# Autodesk Inventor assembly: outsideHand
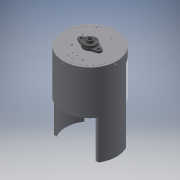
[picture p0: Inventor's stored thumbnail of the model, 180x180]
Saved by Autodesk Inventor 2016 (Build 200138000, 138)
## iProperties
Created: 2016-11-12
Part Number: outsideHand
Material: 一般
Document SubType Name: Assembly
Designer: Daisuke
Author: Daisuke
## Documents named in this file (5)
- C:\Users\Daisuke\Documents\GitHub\CAD\Hand\ver1\outsideHand.iam
- C:\Users\Daisuke\Documents\GitHub\CAD\Hand\ver1\UFL08 -Housing.ipt
- C:\Users\Daisuke\Documents\GitHub\CAD\Hand\ver1\UltrasonicDistanceSencor.ipt
- C:\Users\Daisuke\Documents\GitHub\CAD\Hand\ver1\outsideBottom.ipt
- C:\Users\Daisuke\Documents\GitHub\CAD\Hand\ver1\outsideCover.iam
## Components (4 placed, 4 different names)
1. UFL08 -Housing:1 — 挿入:2, 挿入:3
2. UltrasonicDistanceSencor:1 — 挿入:4, 挿入:5
3. outsideBottom:1 — 挿入:1, 挿入:2, 挿入:3, 挿入:4, 挿入:5, メイト:1
4. outsideCover:1 [sub-assembly] — 挿入:1, メイト:1
## Relationships (6: Insert 5, Mate 1)
- 挿入:1 [Insert]: outsideBottom:1 ↔ outsideCover:1
- 挿入:2 [Insert]: UFL08 -Housing:1 ↔ outsideBottom:1
- 挿入:3 [Insert]: UFL08 -Housing:1 ↔ outsideBottom:1
- 挿入:4 [Insert]: UltrasonicDistanceSencor:1 ↔ outsideBottom:1
- 挿入:5 [Insert]: UltrasonicDistanceSencor:1 ↔ outsideBottom:1
- メイト:1 [Mate]: outsideBottom:1 ↔ outsideCover:1
